# Autodesk Inventor assembly: BodyTop
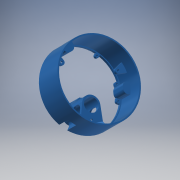
[picture p0: Inventor's stored thumbnail of the model, 180x180]
Saved by Autodesk Inventor 2019.1 (Build 231200000, 200)
## iProperties
Created: 2018-11-28
Part Number: BodyTop
Material: Generisch
Document SubType Name: Assembly
Designer: JochenAlt
Author: JochenAlt
## Documents named in this file (3)
- D:\Projects\Ondine\stl\Body\BodyTop.iam
- D:\Projects\Ondine\CAD\DriveChainEnclosure V3.ipt
- D:\Projects\Ondine\CAD\LegMotorHolder.ipt
## Components (2 placed, 2 different names)
1. DriveChainEnclosure:1 — Passend:1, Passend:2, Passend:3
2. LegMotorHolder:1 — Passend:1, Passend:2, Passend:3
## Relationships (3: Mate 3)
- Passend:1 [Mate]: DriveChainEnclosure:1 ↔ LegMotorHolder:1
- Passend:2 [Mate]: DriveChainEnclosure:1 ↔ LegMotorHolder:1
- Passend:3 [Mate]: DriveChainEnclosure:1 ↔ LegMotorHolder:1
